# Autodesk Inventor assembly: Bumper Assem Full
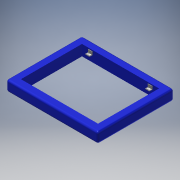
[picture p0: Inventor's stored thumbnail of the model, 180x180]
Saved by Autodesk Inventor 2019 (Build 230136000, 136)
## iProperties
Created: 2018-11-17
Part Number: Bumper Assem Full
Document SubType Name: Assembly
Designer: maste
Author: maste
## Documents named in this file (3)
- D:\Summer Drive Base V1\Summer Drivebase\Bumper Assem Full.iam
- D:\Summer Drive Base V1\Summer Drivebase\Wrap-Around Bumpers.ipt
- D:\Summer Drive Base V1\Summer Drivebase\Bumper Attachment Assembly.iam
## Components (5 placed, 2 different names)
1. Wrap-Around Bumpers:1 — Mate:1, Mate:2, Mate:3, Mate:4, Mate:5, Mate:6, Mate:7, Mate:8, Mate:9, Mate:10, Mate:11, Mate:12
2. Bumper Attachment Assembly:1 [sub-assembly] — Mate:1, Mate:2, Mate:3
3. Bumper Attachment Assembly:2 [sub-assembly] — Mate:4, Mate:5, Mate:6
4. Bumper Attachment Assembly:3 [sub-assembly] — Mate:7, Mate:8, Mate:9
5. Bumper Attachment Assembly:4 [sub-assembly] — Mate:10, Mate:11, Mate:12
## Relationships (12: Mate 12)
- Mate:1: Wrap-Around Bumpers:1 ↔ Bumper Attachment Assembly:1
- Mate:2: Wrap-Around Bumpers:1 ↔ Bumper Attachment Assembly:1
- Mate:3: Wrap-Around Bumpers:1 ↔ Bumper Attachment Assembly:1
- Mate:4: Wrap-Around Bumpers:1 ↔ Bumper Attachment Assembly:2
- Mate:5: Wrap-Around Bumpers:1 ↔ Bumper Attachment Assembly:2
- Mate:6: Wrap-Around Bumpers:1 ↔ Bumper Attachment Assembly:2
- Mate:7: Wrap-Around Bumpers:1 ↔ Bumper Attachment Assembly:3
- Mate:8: Wrap-Around Bumpers:1 ↔ Bumper Attachment Assembly:3
- Mate:9: Wrap-Around Bumpers:1 ↔ Bumper Attachment Assembly:3
- Mate:10: Wrap-Around Bumpers:1 ↔ Bumper Attachment Assembly:4
- Mate:11: Wrap-Around Bumpers:1 ↔ Bumper Attachment Assembly:4
- Mate:12: Wrap-Around Bumpers:1 ↔ Bumper Attachment Assembly:4
